# Autodesk Inventor assembly: WheelieBar Red Alliance
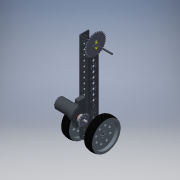
[picture p0: Inventor's stored thumbnail of the model, 180x180]
Saved by Autodesk Inventor 2016 (Build 200138000, 138)
## iProperties
Created: 2015-12-21
Part Number: WheelieBar Red Alliance
Document SubType Name: Assembly
Designer: tbloo
Author: tbloo
## Documents named in this file (15)
- C:\Users\tbloo\Documents\GitHub\phi_robotics\3d-models\FTC_Tetrix_KOP_Block_Party\Tim Bloot Designs\JAr JaR Bot\WheelieBar Red Alliance.iam
- C:\Users\tbloo\Documents\GitHub\phi_robotics\3d-models\FTC_Tetrix_KOP_Block_Party\Tetrix_Kit_FTC\Autodesk Inventor Files\tetrix_c_channel-4.ipt
- C:\Users\tbloo\Documents\GitHub\phi_robotics\3d-models\FTC_Tetrix_KOP_Block_Party\Tetrix_Kit_FTC\Autodesk Inventor Files\tetrix_axle_lock.iam
- C:\Users\tbloo\Documents\GitHub\phi_robotics\3d-models\FTC_Tetrix_KOP_Block_Party\Tetrix_Kit_FTC\Autodesk Inventor Files\tetrix_axle.ipt
- C:\Users\tbloo\Documents\GitHub\phi_robotics\3d-models\FTC_Tetrix_KOP_Block_Party\Tetrix_Kit_FTC\Autodesk Inventor Files\tetrix_chain_gear-32t.ipt
- C:\Users\tbloo\Documents\GitHub\phi_robotics\3d-models\FTC_Tetrix_KOP_Block_Party\Tetrix_Kit_FTC\Autodesk Inventor Files\tetrix_chain_gear-16t.ipt
- C:\Users\tbloo\Documents\GitHub\phi_robotics\3d-models\FTC_Tetrix_KOP_Block_Party\Tetrix_Kit_FTC\Autodesk Inventor Files\tetrix_739092_2012.iam
- C:\Users\tbloo\Documents\GitHub\phi_robotics\3d-models\FTC_Tetrix_KOP_Block_Party\Tetrix_Kit_FTC\Autodesk Inventor Files\tetrix_motor_mount-old.ipt
- C:\Users\tbloo\Documents\GitHub\phi_robotics\3d-models\FTC_Tetrix_KOP_Block_Party\Tetrix_Kit_FTC\Autodesk Inventor Files\tetrix_screw.ipt
- C:\Users\tbloo\Documents\GitHub\phi_robotics\3d-models\FTC_Tetrix_KOP_Block_Party\Tetrix_Kit_FTC\Autodesk Inventor Files\tetrix_axle_spacer-small.ipt
- C:\Users\tbloo\Documents\GitHub\phi_robotics\3d-models\FTC_Tetrix_KOP_Block_Party\Tetrix_Kit_FTC\Autodesk Inventor Files\tetrix_bushing.ipt
- C:\Users\tbloo\Documents\GitHub\phi_robotics\3d-models\FTC_Tetrix_KOP_Block_Party\Tetrix_Kit_FTC\Autodesk Inventor Files\tetrix_wheel.ipt
- C:\Users\tbloo\Documents\GitHub\phi_robotics\3d-models\FTC_Tetrix_KOP_Block_Party\Tetrix_Kit_FTC\Autodesk Inventor Files\tetrix_axle_spacer-big.ipt
- C:\Users\tbloo\Documents\GitHub\phi_robotics\3d-models\FTC_Tetrix_KOP_Block_Party\Tetrix_Kit_FTC\Autodesk Inventor Files\tetrix_motor.iam
- C:\Users\tbloo\Documents\GitHub\phi_robotics\3d-models\FTC_Tetrix_KOP_Block_Party\Tetrix_Kit_FTC\Autodesk Inventor Files\tetrix_maxle_lock.iam
## Components (26 placed, 14 different names)
1. tetrix_c_channel-4:1 — Rigid:18, Rigid:19, Rigid:20, Rotational:5, Rotational:7, Rigid:21
2. tetrix_axle_lock:1 [sub-assembly]
3. tetrix_axle:1
4. tetrix_axle:2
5. tetrix_chain_gear-32t:1 — Rigid:18
6. tetrix_chain_gear-16t:1
7. tetrix_739092_2012:1 [sub-assembly]
8. tetrix_axle_lock:2 [sub-assembly] — Rigid:20
9. tetrix_screw:1
10. tetrix_screw:2
11. tetrix_axle_spacer-small:1
12. tetrix_bushing:1 — Rigid:19
13. tetrix_wheel:1
14. tetrix_wheel:2 — Rotational:6
15. tetrix_axle_lock:3 [sub-assembly]
16. tetrix_screw:3
17. tetrix_screw:4
18. tetrix_axle_spacer-small:2
19. tetrix_bushing:2 — Rotational:5, Rotational:8
20. tetrix_bushing:3 — Rotational:7
21. tetrix_axle_lock:4 [sub-assembly]
22. tetrix_axle_spacer-big:1 — Rotational:6, Rotational:8
23. tetrix_motor_mount-old:1 — Rigid:21, Rotational:9
24. tetrix_motor:1 [sub-assembly] — Rotational:9, Rigid:23
25. tetrix_chain_gear-16t:2
26. tetrix_maxle_lock:1 [sub-assembly] — Rigid:23
## Relationships (25: WeldJoint 20, RevoluteJoint 5)
- [WeldJoint]: tetrix_chain_gear-32t:1 ↔ tetrix_screw:1
- [WeldJoint]: tetrix_chain_gear-32t:1 ↔ tetrix_screw:2
- [WeldJoint]: tetrix_chain_gear-32t:1 ↔ tetrix_axle_spacer-small:1
- [WeldJoint]: tetrix_739092_2012:1 ↔ tetrix_bushing:1
- [WeldJoint]: tetrix_axle:2 ↔ tetrix_739092_2012:1
- [WeldJoint]: tetrix_axle_lock:1 ↔ tetrix_wheel:1
- [WeldJoint]: tetrix_chain_gear-16t:1 ↔ tetrix_axle_lock:3
- [WeldJoint]: tetrix_axle:1 ↔ tetrix_wheel:1
- [WeldJoint]: tetrix_axle_lock:1 ↔ tetrix_axle_lock:3
- [WeldJoint]: tetrix_chain_gear-16t:1 ↔ tetrix_screw:3
- [WeldJoint]: tetrix_chain_gear-16t:1 ↔ tetrix_screw:4
- [WeldJoint]: tetrix_chain_gear-16t:1 ↔ tetrix_axle_spacer-small:2
- [WeldJoint]: tetrix_wheel:2 ↔ tetrix_axle_lock:4
- [WeldJoint] (-25.5 mm): tetrix_axle:1 ↔ tetrix_wheel:2
- Rigid:18 [WeldJoint]: tetrix_c_channel-4:1 ↔ tetrix_chain_gear-32t:1
- Rigid:19 [WeldJoint]: tetrix_c_channel-4:1 ↔ tetrix_bushing:1
- Rigid:20 [WeldJoint]: tetrix_c_channel-4:1 ↔ tetrix_axle_lock:2
- Rotational:5 [RevoluteJoint]: tetrix_c_channel-4:1 ↔ tetrix_bushing:2
- Rotational:6 [RevoluteJoint]: tetrix_wheel:2 ↔ tetrix_axle_spacer-big:1
- Rotational:7 [RevoluteJoint]: tetrix_c_channel-4:1 ↔ tetrix_bushing:3
- Rotational:8 [RevoluteJoint]: tetrix_bushing:2 ↔ tetrix_axle_spacer-big:1
- Rigid:21 [WeldJoint]: tetrix_c_channel-4:1 ↔ tetrix_motor_mount-old:1
- Rotational:9 [RevoluteJoint]: tetrix_motor_mount-old:1 ↔ tetrix_motor:1
- [WeldJoint]: tetrix_chain_gear-16t:2 ↔ tetrix_maxle_lock:1
- Rigid:23 [WeldJoint] (-23 mm): tetrix_motor:1 ↔ tetrix_maxle_lock:1
